# Autodesk Inventor assembly: rack_and_pinion
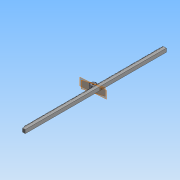
[picture p0: Inventor's stored thumbnail of the model, 180x180]
Saved by Autodesk Inventor 2015 (Build 190159000, 159)
## iProperties
Created: 2014-09-02
Part Number: rack_and_pinion
Document SubType Name: Assembly
Designer: shohei
Author: shohei
## Documents named in this file (3)
- C:\Users\shohei\Documents\Inventor\PlasmaCNCrev3\Workspaces\Workspace\rack_and_pinion_X.iam
- C:\Users\shohei\Documents\Inventor\PlasmaCNCrev3\Workspaces\Workspace\rack_and_pinion\Design Accelerator\Spur Gears1.iam
- C:\Users\shohei\Documents\Inventor\PlasmaCNCrev3\Workspaces\Workspace\rack_X.ipt
## Components (2 placed, 2 different names)
1. Spur Gears:1 [sub-assembly] — Mate:1, Mate:2, Tangent:1, Mate:3, Angle:9, Rotation/Translation:1
2. rack_X:1 — Angle:8, Tangent:1, Flush:1, Rotation/Translation:1
## Relationships (9: Mate 3, Angle 3, Tangent 1, Flush 1, RelateRotateTranslate 1)
- Mate:1: Spur Gears:1
- Mate:2: Spur Gears:1
- Angle:8 (0 deg): rack_X:1
- Tangent:1: Spur Gears:1 ↔ rack_X:1
- Flush:1 (-28.31 mm): rack_X:1
- Mate:3: Spur Gears:1
- Angle:9 (12 deg): Spur Gears:1
- Rotation/Translation:1 [RelateRotateTranslate] (47.1239 mm): Spur Gears:1 ↔ rack_X:1
- Angle:10 (0 deg)
